# Autodesk Inventor assembly: NEMA 17 with T5 Pulley
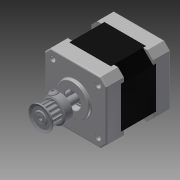
[picture p0: Inventor's stored thumbnail of the model, 180x180]
Saved by Autodesk Inventor 2015 (Build 190159000, 159)
## iProperties
Created: 2017-01-04
Part Number: NEMA 17 with T5 Pulley
Document SubType Name: Assembly
Designer: Ernest
Title: NEMA 17 with T5 Pulley.STEP
Description: STEP AP203
Creation Date: 2013-02-23
Sending System: SolidWorks 2012
Preprocessor: SwSTEP 2.0
Author: Ernest
## Documents named in this file (9)
- C:\Users\Ernest\Documents\Capstone-Project\doc\CAD\Imported Components\NEMA 17 with T5 Pulley\NEMA 17 with T5 Pulley.iam
- C:\Users\Ernest\Documents\Capstone-Project\doc\CAD\Imported Components\NEMA 17 with T5 Pulley\Base.ipt
- C:\Users\Ernest\Documents\Capstone-Project\doc\CAD\Imported Components\NEMA 17 with T5 Pulley\Cuerpo.ipt
- C:\Users\Ernest\Documents\Capstone-Project\doc\CAD\Imported Components\NEMA 17 with T5 Pulley\Tapa.ipt
- C:\Users\Ernest\Documents\Capstone-Project\doc\CAD\Imported Components\NEMA 17 with T5 Pulley\pan cross head_am_B18.6.7M - M3 x 0.5 x 5 Type I Cross Recessed PHMS --5N.ipt
- C:\Users\Ernest\Documents\Capstone-Project\doc\CAD\Imported Components\NEMA 17 with T5 Pulley\Eje.ipt
- C:\Users\Ernest\Documents\Capstone-Project\doc\CAD\Imported Components\NEMA 17 with T5 Pulley\instrument ball bearing_68_am_AFBMA 12.1.4.1 - 0050-11 - 10,SI,NC,10_68.ipt
- C:\Users\Ernest\Documents\Capstone-Project\doc\CAD\Imported Components\NEMA 17 with T5 Pulley\socket button head cap screw_am_B18.3.4M - 3 x 0.5 x 5 SBHCS --N.ipt
- C:\Users\Ernest\Documents\Capstone-Project\doc\CAD\Imported Components\NEMA 17 with T5 Pulley\T5 Pulley.ipt
## Components (12 placed, 12 different names)
1. Base_1 — Mate:1, Flush:1, Flush:2, Flush:3, Flush:4, Mate:7, Mate:8, Mate:9, Mate:10, Mate:11, Mate:12, Mate:13
2. Cuerpo_2 — Flush:3, Flush:4, Mate:2
3. Tapa_3 — Mate:1, Flush:1, Flush:2, Mate:2, Flush:5, Mate:4, Mate:5, Mate:6
4. pan cross head_am_B18.6.7M - M3 x 0.5 x 5 Type I Cross Recessed PHMS --5N_4 — Mate:9, Flush:8, Mate:13
5. pan cross head_am_B18.6.7M - M3 x 0.5 x 5 Type I Cross Recessed PHMS --5N_5 — Mate:10, Flush:6
6. pan cross head_am_B18.6.7M - M3 x 0.5 x 5 Type I Cross Recessed PHMS --5N_6 — Mate:12, Flush:6, Flush:7
7. pan cross head_am_B18.6.7M - M3 x 0.5 x 5 Type I Cross Recessed PHMS --5N_7 — Mate:11, Flush:7, Flush:8
8. Eje_8 — Flush:5, Mate:4, Mate:14, Flush:9
9. instrument ball bearing_68_am_AFBMA 12.1.4.1 - 0050-11 - 10,SI,NC,10_68_9 — Mate:5, Mate:6
10. instrument ball bearing_68_am_AFBMA 12.1.4.1 - 0050-11 - 10,SI,NC,10_68_10 — Mate:7, Mate:8
11. socket button head cap screw_am_B18.3.4M - 3 x 0.5 x 5 SBHCS --N_11 — Mate:3, Tangent:1
12. T5 Pulley_12 — Mate:3, Tangent:1, Mate:14, Flush:9
## Relationships (24: Mate 14, Flush 9, Tangent 1)
- Mate:1 (-44 mm): Base_1 ↔ Tapa_3
- Flush:1: Base_1 ↔ Tapa_3
- Flush:2: Base_1 ↔ Tapa_3
- Flush:3: Base_1 ↔ Cuerpo_2
- Flush:4: Base_1 ↔ Cuerpo_2
- Mate:2: Cuerpo_2 ↔ Tapa_3
- Mate:3: socket button head cap screw_am_B18.3.4M - 3 x 0.5 x 5 SBHCS --N_11 ↔ T5 Pulley_12
- Tangent:1: socket button head cap screw_am_B18.3.4M - 3 x 0.5 x 5 SBHCS --N_11 ↔ T5 Pulley_12
- Flush:5 (-22 mm): Tapa_3 ↔ Eje_8
- Mate:4: Tapa_3 ↔ Eje_8
- Mate:5: Tapa_3 ↔ instrument ball bearing_68_am_AFBMA 12.1.4.1 - 0050-11 - 10,SI,NC,10_68_9
- Mate:6: Tapa_3 ↔ instrument ball bearing_68_am_AFBMA 12.1.4.1 - 0050-11 - 10,SI,NC,10_68_9
- Mate:7: Base_1 ↔ instrument ball bearing_68_am_AFBMA 12.1.4.1 - 0050-11 - 10,SI,NC,10_68_10
- Mate:8: Base_1 ↔ instrument ball bearing_68_am_AFBMA 12.1.4.1 - 0050-11 - 10,SI,NC,10_68_10
- Mate:9: Base_1 ↔ pan cross head_am_B18.6.7M - M3 x 0.5 x 5 Type I Cross Recessed PHMS --5N_4
- Mate:10: Base_1 ↔ pan cross head_am_B18.6.7M - M3 x 0.5 x 5 Type I Cross Recessed PHMS --5N_5
- Mate:11: Base_1 ↔ pan cross head_am_B18.6.7M - M3 x 0.5 x 5 Type I Cross Recessed PHMS --5N_7
- Mate:12: Base_1 ↔ pan cross head_am_B18.6.7M - M3 x 0.5 x 5 Type I Cross Recessed PHMS --5N_6
- Flush:6: pan cross head_am_B18.6.7M - M3 x 0.5 x 5 Type I Cross Recessed PHMS --5N_5 ↔ pan cross head_am_B18.6.7M - M3 x 0.5 x 5 Type I Cross Recessed PHMS --5N_6
- Flush:7: pan cross head_am_B18.6.7M - M3 x 0.5 x 5 Type I Cross Recessed PHMS --5N_6 ↔ pan cross head_am_B18.6.7M - M3 x 0.5 x 5 Type I Cross Recessed PHMS --5N_7
- Flush:8: pan cross head_am_B18.6.7M - M3 x 0.5 x 5 Type I Cross Recessed PHMS --5N_4 ↔ pan cross head_am_B18.6.7M - M3 x 0.5 x 5 Type I Cross Recessed PHMS --5N_7
- Mate:13: Base_1 ↔ pan cross head_am_B18.6.7M - M3 x 0.5 x 5 Type I Cross Recessed PHMS --5N_4
- Mate:14: Eje_8 ↔ T5 Pulley_12
- Flush:9: Eje_8 ↔ T5 Pulley_12
